# Autodesk Inventor assembly: 71. Шестерня первой передачи
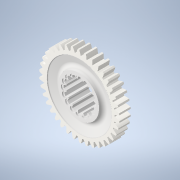
[picture p0: Inventor's stored thumbnail of the model, 180x180]
Saved by Autodesk Inventor 2021 (Build 250183000, 183)
## iProperties
Created: 2021-03-23
Part Number: 71. Шестерня первой передачи
Document SubType Name: Assembly
Designer: Данил
Author: Данил
## Documents named in this file (3)
- C:\Users\Данил\Desktop\Коробка передач\Детали\71. Шестерня первой передачи.iam
- C:\Users\Данил\Desktop\Коробка передач\Детали\71. Шестерня первой передачи.ipt
- C:\Users\Данил\Desktop\Коробка передач\Детали\71. Шестерня первой передачи\Мастер проектирования\Цилиндрическое зубчатое зацепление1.iam
## Components (2 placed, 2 different names)
1. 71. Шестерня первой передачи:1 — Совмещение:1, Заподлицо:1
2. Цилиндрическое зубчатое зацепление:1 [sub-assembly] — Совмещение:1, Заподлицо:1
## Relationships (2: Mate 1, Flush 1)
- Совмещение:1 [Mate]: 71. Шестерня первой передачи:1 ↔ Цилиндрическое зубчатое зацепление:1
- Заподлицо:1 [Flush]: 71. Шестерня первой передачи:1 ↔ Цилиндрическое зубчатое зацепление:1
